# Autodesk Inventor assembly: Rigid_Coupler_5mm_8mm
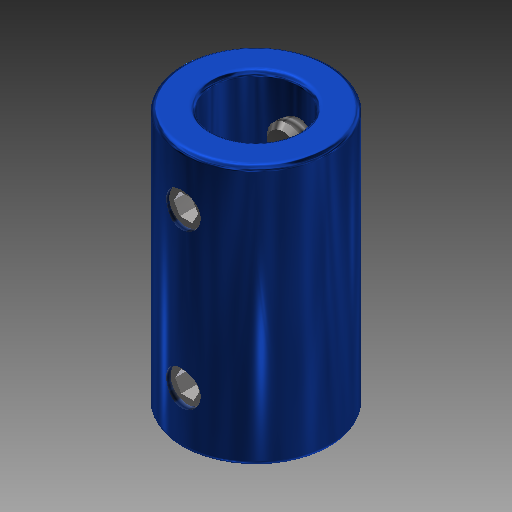
[picture p0: Inventor's stored thumbnail of the model, 512x512]
Saved by Autodesk Inventor 2019 (Build 230136000, 136)
## iProperties
Created: 2018-09-15
Part Number: Rigid_Coupler_5mm_8mm
Document SubType Name: Assembly
Designer: Ax
Mass: 8.79814 g
Surface Area: 22.37 cm^2
Volume: 2.94596 cm^3
Density: 2.98651 g/cm^3
Author: Ax
## Documents named in this file (3)
- C:\Users\Ax\Google Drive\Inventor\Library\Rigid_Coupler_5mm_8mm.iam
- C:\Users\Ax\Google Drive\Inventor\Library\Rigid_Coupler.ipt
- C:\Users\Ax\Google Drive\Autodesk\Content Center Files\R2017\en-US\ANSI B18.3.6M(05)\ANSI B18.3.6M - M4x0.7 x 4(1).ipt
## Components (5 placed, 2 different names)
1. Rigid_Coupler:1 — Rigid:2, Rigid:3, Rigid:4, Rigid:5
2. Forged Hexagon Socket Set Screw - Flat Point - Metric M4x0.7 x 4:1 — Rigid:2
3. Forged Hexagon Socket Set Screw - Flat Point - Metric M4x0.7 x 4:2 — Rigid:5
4. Forged Hexagon Socket Set Screw - Flat Point - Metric M4x0.7 x 4:3 — Rigid:3
5. Forged Hexagon Socket Set Screw - Flat Point - Metric M4x0.7 x 4:4 — Rigid:4
## Relationships (4: WeldJoint 4)
- Rigid:2 [WeldJoint]: Rigid_Coupler:1 ↔ Forged Hexagon Socket Set Screw - Flat Point - Metric M4x0.7 x 4:1
- Rigid:3 [WeldJoint] (0.75 mm): Rigid_Coupler:1 ↔ Forged Hexagon Socket Set Screw - Flat Point - Metric M4x0.7 x 4:3
- Rigid:4 [WeldJoint] (-0.75 mm): Rigid_Coupler:1 ↔ Forged Hexagon Socket Set Screw - Flat Point - Metric M4x0.7 x 4:4
- Rigid:5 [WeldJoint]: Rigid_Coupler:1 ↔ Forged Hexagon Socket Set Screw - Flat Point - Metric M4x0.7 x 4:2
